# Autodesk Inventor assembly: 000-base_wheel-v3
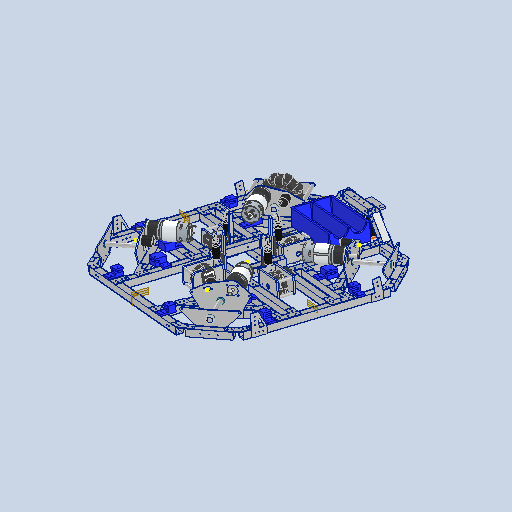
[picture p0: Inventor's stored thumbnail of the model, 512x512]
Saved by Autodesk Inventor 2025.2 (Build 292293000, 293)
## iProperties
Created: 2025-04-01
Part Number: 000-base_wheel-v3
Document SubType Name: Assembly
Designer: haruy
Author: haruy
## Documents named in this file (28)
- C:\Users\haruy\Documents\ロボコン\NHK2025\cad\nagahisa\base_weel\000-base_wheel-v3.iam
- C:\Users\haruy\Documents\ロボコン\NHK2025\cad\nagahisa\base_weel\base_weel-v3-ASP-Base.ipt
- C:\Users\haruy\Documents\ロボコン\NHK2025\cad\nagahisa\base_weel\base_weel-v3-Plate-1.ipt
- C:\Users\haruy\Documents\ロボコン\NHK2025\cad\nagahisa\base_weel\base_weel-v3-Plate-2.ipt
- C:\Users\haruy\Documents\ロボコン\NHK2025\cad\nagahisa\base_weel\takagi_weel\Workspaces\作業スペース\takagi\omuni_wheel_ver3.0\parts\frequently used parts\モーター\RS775\rs775_4.iam
- C:\Users\haruy\Documents\ロボコン\NHK2025\cad\000_parts\エンコーダー\encoder v2.ipt
- C:\Users\haruy\Documents\ロボコン\NHK2025\cad\nagahisa\odom\odom_v1_Plate_5.ipt
- C:\Users\haruy\Documents\ロボコン\NHK2025\cad\nagahisa\odom\000-odom-v1.iam
- C:\Users\haruy\Documents\ロボコン\NHK2025\cad\nagahisa\odom\odom_v1_Plate_6.ipt
- C:\Users\haruy\Documents\ロボコン\NHK2025\cad\nagahisa\base_weel\base_weel-v3-Plate-3.ipt
- C:\Users\haruy\Documents\ロボコン\NHK2025\cad\nagahisa\base_weel\base_weel-v3-Plate-4.ipt
- C:\Users\haruy\Documents\ロボコン\NHK2025\cad\nagahisa\base_weel\base_weel-v3-Plate-5.ipt
- C:\Users\haruy\Documents\ロボコン\NHK2025\cad\nagahisa\base_weel\base_weel-v3-Plate-6.ipt
- C:\Users\haruy\Documents\ロボコン\NHK2025\cad\nagahisa\dribl\R2-Rzvector\TH22_bearing_12_18_19.5_sn.ipt
- C:\Users\haruy\Documents\ロボコン\NHK2025\cad\nagahisa\base_weel\SCBRJ12-15.iam
- C:\Users\haruy\Documents\ロボコン\NHK2025\cad\nagahisa\base_weel\base_weel-v3-Shaft-1.ipt
- C:\Users\haruy\Documents\ロボコン\NHK2025\cad\nagahisa\base_weel\takagi_weel\Workspaces\作業スペース\takagi\omuni_wheel_ver3.0\parts\frequently used parts\タイヤ\omni wheel\100mm wheel\100mm omuniwheel_MIR1.iam
- C:\Users\haruy\Documents\ロボコン\NHK2025\cad\nagahisa\base_weel\base_weel-v3-Shaft-2.ipt
- C:\Users\haruy\Documents\ロボコン\NHK2025\cad\nagahisa\base_weel\base_weel-v3-Plate-7.ipt
- C:\Users\haruy\Documents\ロボコン\NHK2025\cad\nagahisa\base_weel\roja-v1-3DP-lipo-box.ipt
- C:\Users\haruy\Documents\ロボコン\NHK2025\cad\nagahisa\base_weel\base_weel-v3-3DP-1.ipt
- C:\Users\haruy\Documents\ロボコン\NHK2025\cad\nagahisa\base_weel\base_weel-v3-3DP-2.ipt
- C:\Users\haruy\Documents\ロボコン\NHK2025\cad\nagahisa\base_weel\base_weel-v3-Plate-8.ipt
- C:\Users\haruy\Documents\ロボコン\NHK2025\cad\000_parts\センサー\LiDAR_true.iam
- C:\Users\haruy\Documents\ロボコン\NHK2025\cad\nagahisa\base_weel\base_weel-v3-Plate-9.ipt
- C:\Users\haruy\Documents\ロボコン\NHK2025\cad\nagahisa\base_weel\base_weel-v3-Plate-10.ipt
- C:\Users\haruy\Documents\ロボコン\NHK2025\cad\nagahisa\dribl\dribl-v1-Plate-9.ipt
- C:\Users\haruy\Documents\ロボコン\NHK2025\cad\nagahisa\dribl\dribl-v3-Plate-5.ipt
## Components (93 placed, 27 different names)
1. base_weel-v3-ASP-Base:1 — 挿入:1, 挿入:2, 挿入:3, 挿入:4, 挿入:5, 挿入:6, 挿入:7, 挿入:8, 挿入:9, 挿入:10, 挿入:11, 挿入:12, 挿入:13, 挿入:14, 挿入:15, 挿入:16, 挿入:25, 挿入:26, 挿入:27, 挿入:28, 挿入:35, 挿入:36, 挿入:37, 挿入:38, 挿入:45, 挿入:46, 挿入:47, 挿入:48, 挿入:49, 挿入:50, 挿入:51, 挿入:52, 挿入:53, 挿入:54, 挿入:55, 挿入:56, 挿入:57, 挿入:58, 挿入:59, 挿入:60, 挿入:61, 挿入:62, 挿入:63, 挿入:64, 挿入:65, 挿入:66, 挿入:67, 挿入:68, 挿入:69, 挿入:70, 挿入:71, 挿入:72, 挿入:73, 挿入:74, 挿入:75, 挿入:76, 挿入:77, 挿入:78, 挿入:79, 挿入:80, 挿入:81, 挿入:82, 挿入:87, 挿入:88, 挿入:89, 挿入:90, 挿入:91, 挿入:92, 挿入:93, 挿入:94, 挿入:95, 挿入:96, 挿入:97, 挿入:98, 挿入:99, 挿入:100, 角度:1, 挿入:124, 挿入:125, 挿入:126, 挿入:127, 挿入:128, 挿入:129, 挿入:130, 挿入:131, 挿入:132, 挿入:133, 挿入:134, 挿入:135, 挿入:136, 挿入:137, 挿入:138, 挿入:139, 挿入:140, 挿入:141, 挿入:142, 挿入:143, 挿入:146, 挿入:147, 挿入:148, 挿入:149, 挿入:150, 挿入:151, 挿入:152, 挿入:153, 挿入:154, 挿入:155, 挿入:156, 挿入:157, 挿入:158, 挿入:159, 挿入:160, 挿入:161
2. base_weel-v3-Plate-1:1 — 挿入:1, 挿入:2, 挿入:108
3. base_weel-v3-Plate-1:2 — 挿入:3, 挿入:4, 挿入:105
4. base_weel-v3-Plate-1:3 — 挿入:7, 挿入:8, 挿入:101
5. base_weel-v3-Plate-1:4 — 挿入:5, 挿入:6, 挿入:103
6. base_weel-v3-Plate-2:1 — 挿入:9, 挿入:10, 挿入:17, 挿入:23, 挿入:104
7. base_weel-v3-Plate-2:2 — 挿入:11, 挿入:12, 挿入:20, 挿入:21, 挿入:107
8. base_weel-v3-Plate-2:3 — 挿入:13, 挿入:14, 挿入:18, 挿入:24, 挿入:102, 挿入:122, 挿入:123
9. base_weel-v3-Plate-2:4 — 挿入:15, 挿入:16, 挿入:19, 挿入:22, 挿入:106
10. rs775_4:1 [sub-assembly] — 挿入:17
11. rs775_4:2 [sub-assembly] — 挿入:18
12. rs775_4:3 [sub-assembly] — 挿入:19
13. rs775_4:4 [sub-assembly] — 挿入:20
14. encoder v2:1 — 挿入:21
15. encoder v2:2 — 挿入:22
16. encoder v2:3 — 挿入:23
17. encoder v2:4 — 挿入:24
18. odom_v1_Plate_5:1 — 挿入:26, 挿入:28, 挿入:29, 挿入:30, 挿入:31
19. odom_v1_Plate_5:2 — 挿入:25, 挿入:27, 挿入:32, 挿入:33, 挿入:34
20. 000-odom-v1:1 [sub-assembly] — 挿入:29, 挿入:30, 挿入:31
21. 000-odom-v1:2 [sub-assembly] — 挿入:32, 挿入:33, 挿入:34
22. odom_v1_Plate_6:1 — 挿入:35, 挿入:36, 挿入:39, 挿入:40, 挿入:41
23. odom_v1_Plate_6:2 — 挿入:37, 挿入:38, 挿入:42, 挿入:43, 挿入:44
24. 000-odom-v1:3 [sub-assembly] — 挿入:39, 挿入:40, 挿入:41
25. 000-odom-v1:4 [sub-assembly] — 挿入:42, 挿入:43, 挿入:44
26. base_weel-v3-Plate-3:1 — 挿入:45, 挿入:46
27. base_weel-v3-Plate-3:2 — 挿入:47, 挿入:48
28. base_weel-v3-Plate-3:3 — 挿入:49, 挿入:50
29. base_weel-v3-Plate-3:4 — 挿入:51, 挿入:52
30. base_weel-v3-Plate-3:5 — 挿入:53, 挿入:54
31. base_weel-v3-Plate-3:6 — 挿入:57, 挿入:58
32. base_weel-v3-Plate-3:7 — 挿入:59, 挿入:60
33. base_weel-v3-Plate-3:8 — 挿入:55, 挿入:56
34. base_weel-v3-Plate-4:1 — 挿入:61, 挿入:62
35. base_weel-v3-Plate-4:2 — 挿入:63, 挿入:64
36. base_weel-v3-Plate-4:3 — 挿入:67, 挿入:68
37. base_weel-v3-Plate-4:4 — 挿入:65, 挿入:66
38. base_weel-v3-Plate-4:5 — 挿入:71, 挿入:72
39. base_weel-v3-Plate-4:6 — 挿入:73, 挿入:74
40. base_weel-v3-Plate-4:7 — 挿入:69, 挿入:70
41. base_weel-v3-Plate-4:8 — 挿入:75, 挿入:76
42. base_weel-v3-Plate-5:1 — 挿入:77, 挿入:78
43. base_weel-v3-Plate-5:2 — 挿入:79, 挿入:80
44. base_weel-v3-Plate-5:3 — 挿入:81, 挿入:82
45. base_weel-v3-Plate-5:6 — 挿入:87, 挿入:88
46. base_weel-v3-Plate-5:7 — 挿入:89, 挿入:90
47. base_weel-v3-Plate-5:8 — 挿入:91, 挿入:92
48. base_weel-v3-Plate-6:1 — 挿入:93, 挿入:94
49. base_weel-v3-Plate-6:2 — 挿入:95, 挿入:96
50. base_weel-v3-Plate-6:3 — 挿入:97, 挿入:98
51. base_weel-v3-Plate-6:4 — 挿入:99, 挿入:100
52. TH22_bearing_12_18_19.5_sn:1 — 挿入:101, 挿入:113, 挿入:121
53. TH22_bearing_12_18_19.5_sn:2 — 挿入:102, 挿入:114
54. TH22_bearing_12_18_19.5_sn:3 — 挿入:104, 挿入:115
55. TH22_bearing_12_18_19.5_sn:4 — 挿入:103, 挿入:116
56. TH22_bearing_12_18_19.5_sn:5 — 挿入:105, 挿入:109
57. TH22_bearing_12_18_19.5_sn:6 — 挿入:107, 挿入:112
58. TH22_bearing_12_18_19.5_sn:7 — 挿入:106, 挿入:110
59. TH22_bearing_12_18_19.5_sn:8 — 挿入:108, 挿入:111
60. SCBRJ12-15:1 [sub-assembly] — 挿入:116, 挿入:120
61. SCBRJ12-15:2 [sub-assembly] — 挿入:112
62. SCBRJ12-15:3 [sub-assembly] — 挿入:115
63. SCBRJ12-15:4 [sub-assembly] — 挿入:109, 挿入:117
64. SCBRJ12-15:5 [sub-assembly] — 挿入:114
65. SCBRJ12-15:6 [sub-assembly] — 挿入:110
66. SCBRJ12-15:7 [sub-assembly] — 挿入:113, 挿入:119
67. SCBRJ12-15:8 [sub-assembly] — 挿入:111, 挿入:118
68. base_weel-v3-Shaft-1:1 — 挿入:117
69. base_weel-v3-Shaft-1:2 — 挿入:118
70. base_weel-v3-Shaft-1:3 — 挿入:119
71. base_weel-v3-Shaft-1:4 — 挿入:120
72. 100mm omuniwheel_MIR1:1 [sub-assembly] — 挿入:121, 角度:1
73. base_weel-v3-Shaft-2:1 — 挿入:122
74. base_weel-v3-Shaft-2:2 — 挿入:123
75. base_weel-v3-Plate-7:1 — 挿入:124, 挿入:125
76. base_weel-v3-Plate-7:2 — 挿入:126, 挿入:127
77. roja-v1-3DP-lipo-box:1 — 挿入:128, 挿入:129
78. base_weel-v3-3DP-1:2 — 挿入:130, 挿入:131
79. base_weel-v3-3DP-1:3 — 挿入:134, 挿入:135
80. base_weel-v3-3DP-1:6 — 挿入:132, 挿入:133
81. base_weel-v3-3DP-2:1 — 挿入:136, 挿入:137
82. base_weel-v3-3DP-2:2 — 挿入:138, 挿入:139
83. base_weel-v3-3DP-2:3 — 挿入:140, 挿入:141
84. base_weel-v3-Plate-8:1 — 挿入:142, 挿入:143, 挿入:144, 挿入:145
85. LiDAR_true:1 [sub-assembly] — 挿入:144, 挿入:145
86. base_weel-v3-Plate-9:1 — 挿入:146, 挿入:147
87. base_weel-v3-Plate-9:2 — 挿入:148, 挿入:149
88. base_weel-v3-Plate-10:1 — 挿入:150, 挿入:151
89. base_weel-v3-Plate-10:2 — 挿入:152, 挿入:153
90. dribl-v1-Plate-9:1 — 挿入:156, 挿入:157
91. dribl-v1-Plate-9:2 — 挿入:154, 挿入:155
92. dribl-v3-Plate-5:1 — 挿入:158, 挿入:159
93. dribl-v3-Plate-5:2 — 挿入:160, 挿入:161
## Relationships (158: Insert 157, Angle 1)
- 挿入:1 [Insert]: base_weel-v3-ASP-Base:1 ↔ base_weel-v3-Plate-1:1
- 挿入:2 [Insert]: base_weel-v3-ASP-Base:1 ↔ base_weel-v3-Plate-1:1
- 挿入:3 [Insert]: base_weel-v3-ASP-Base:1 ↔ base_weel-v3-Plate-1:2
- 挿入:4 [Insert]: base_weel-v3-ASP-Base:1 ↔ base_weel-v3-Plate-1:2
- 挿入:5 [Insert]: base_weel-v3-ASP-Base:1 ↔ base_weel-v3-Plate-1:4
- 挿入:6 [Insert]: base_weel-v3-ASP-Base:1 ↔ base_weel-v3-Plate-1:4
- 挿入:7 [Insert]: base_weel-v3-ASP-Base:1 ↔ base_weel-v3-Plate-1:3
- 挿入:8 [Insert]: base_weel-v3-ASP-Base:1 ↔ base_weel-v3-Plate-1:3
- 挿入:9 [Insert]: base_weel-v3-ASP-Base:1 ↔ base_weel-v3-Plate-2:1
- 挿入:10 [Insert]: base_weel-v3-ASP-Base:1 ↔ base_weel-v3-Plate-2:1
- 挿入:11 [Insert]: base_weel-v3-ASP-Base:1 ↔ base_weel-v3-Plate-2:2
- 挿入:12 [Insert]: base_weel-v3-ASP-Base:1 ↔ base_weel-v3-Plate-2:2
- 挿入:13 [Insert]: base_weel-v3-ASP-Base:1 ↔ base_weel-v3-Plate-2:3
- 挿入:14 [Insert]: base_weel-v3-ASP-Base:1 ↔ base_weel-v3-Plate-2:3
- 挿入:15 [Insert]: base_weel-v3-ASP-Base:1 ↔ base_weel-v3-Plate-2:4
- 挿入:16 [Insert]: base_weel-v3-ASP-Base:1 ↔ base_weel-v3-Plate-2:4
- 挿入:17 [Insert]: base_weel-v3-Plate-2:1 ↔ rs775_4:1
- 挿入:18 [Insert]: base_weel-v3-Plate-2:3 ↔ rs775_4:2
- 挿入:19 [Insert]: base_weel-v3-Plate-2:4 ↔ rs775_4:3
- 挿入:20 [Insert]: base_weel-v3-Plate-2:2 ↔ rs775_4:4
- 挿入:21 [Insert]: base_weel-v3-Plate-2:2 ↔ encoder v2:1
- 挿入:22 [Insert]: base_weel-v3-Plate-2:4 ↔ encoder v2:2
- 挿入:23 [Insert]: base_weel-v3-Plate-2:1 ↔ encoder v2:3
- 挿入:24 [Insert]: base_weel-v3-Plate-2:3 ↔ encoder v2:4
- 挿入:25 [Insert]: base_weel-v3-ASP-Base:1 ↔ odom_v1_Plate_5:2
- 挿入:26 [Insert]: base_weel-v3-ASP-Base:1 ↔ odom_v1_Plate_5:1
- 挿入:27 [Insert]: base_weel-v3-ASP-Base:1 ↔ odom_v1_Plate_5:2
- 挿入:28 [Insert]: base_weel-v3-ASP-Base:1 ↔ odom_v1_Plate_5:1
- 挿入:29 [Insert]: odom_v1_Plate_5:1 ↔ 000-odom-v1:1
- 挿入:30 [Insert]: odom_v1_Plate_5:1 ↔ 000-odom-v1:1
- 挿入:31 [Insert]: odom_v1_Plate_5:1 ↔ 000-odom-v1:1
- 挿入:32 [Insert]: odom_v1_Plate_5:2 ↔ 000-odom-v1:2
- 挿入:33 [Insert]: odom_v1_Plate_5:2 ↔ 000-odom-v1:2
- 挿入:34 [Insert]: odom_v1_Plate_5:2 ↔ 000-odom-v1:2
- 挿入:35 [Insert]: base_weel-v3-ASP-Base:1 ↔ odom_v1_Plate_6:1
- 挿入:36 [Insert]: base_weel-v3-ASP-Base:1 ↔ odom_v1_Plate_6:1
- 挿入:37 [Insert]: base_weel-v3-ASP-Base:1 ↔ odom_v1_Plate_6:2
- 挿入:38 [Insert]: base_weel-v3-ASP-Base:1 ↔ odom_v1_Plate_6:2
- 挿入:39 [Insert]: odom_v1_Plate_6:1 ↔ 000-odom-v1:3
- 挿入:40 [Insert]: odom_v1_Plate_6:1 ↔ 000-odom-v1:3
- 挿入:41 [Insert]: odom_v1_Plate_6:1 ↔ 000-odom-v1:3
- 挿入:42 [Insert]: odom_v1_Plate_6:2 ↔ 000-odom-v1:4
- 挿入:43 [Insert]: odom_v1_Plate_6:2 ↔ 000-odom-v1:4
- 挿入:44 [Insert]: odom_v1_Plate_6:2 ↔ 000-odom-v1:4
- 挿入:45 [Insert]: base_weel-v3-ASP-Base:1 ↔ base_weel-v3-Plate-3:1
- 挿入:46 [Insert]: base_weel-v3-ASP-Base:1 ↔ base_weel-v3-Plate-3:1
- 挿入:47 [Insert]: base_weel-v3-ASP-Base:1 ↔ base_weel-v3-Plate-3:2
- 挿入:48 [Insert]: base_weel-v3-ASP-Base:1 ↔ base_weel-v3-Plate-3:2
- 挿入:49 [Insert]: base_weel-v3-ASP-Base:1 ↔ base_weel-v3-Plate-3:3
- 挿入:50 [Insert]: base_weel-v3-ASP-Base:1 ↔ base_weel-v3-Plate-3:3
- 挿入:51 [Insert]: base_weel-v3-ASP-Base:1 ↔ base_weel-v3-Plate-3:4
- 挿入:52 [Insert]: base_weel-v3-ASP-Base:1 ↔ base_weel-v3-Plate-3:4
- 挿入:53 [Insert]: base_weel-v3-ASP-Base:1 ↔ base_weel-v3-Plate-3:5
- 挿入:54 [Insert]: base_weel-v3-ASP-Base:1 ↔ base_weel-v3-Plate-3:5
- 挿入:55 [Insert]: base_weel-v3-ASP-Base:1 ↔ base_weel-v3-Plate-3:8
- 挿入:56 [Insert]: base_weel-v3-ASP-Base:1 ↔ base_weel-v3-Plate-3:8
- 挿入:57 [Insert]: base_weel-v3-ASP-Base:1 ↔ base_weel-v3-Plate-3:6
- 挿入:58 [Insert]: base_weel-v3-ASP-Base:1 ↔ base_weel-v3-Plate-3:6
- 挿入:59 [Insert]: base_weel-v3-ASP-Base:1 ↔ base_weel-v3-Plate-3:7
- 挿入:60 [Insert]: base_weel-v3-ASP-Base:1 ↔ base_weel-v3-Plate-3:7
- 挿入:61 [Insert]: base_weel-v3-ASP-Base:1 ↔ base_weel-v3-Plate-4:1
- 挿入:62 [Insert]: base_weel-v3-ASP-Base:1 ↔ base_weel-v3-Plate-4:1
- 挿入:63 [Insert]: base_weel-v3-ASP-Base:1 ↔ base_weel-v3-Plate-4:2
- 挿入:64 [Insert]: base_weel-v3-ASP-Base:1 ↔ base_weel-v3-Plate-4:2
- 挿入:65 [Insert]: base_weel-v3-ASP-Base:1 ↔ base_weel-v3-Plate-4:4
- 挿入:66 [Insert]: base_weel-v3-ASP-Base:1 ↔ base_weel-v3-Plate-4:4
- 挿入:67 [Insert]: base_weel-v3-ASP-Base:1 ↔ base_weel-v3-Plate-4:3
- 挿入:68 [Insert]: base_weel-v3-ASP-Base:1 ↔ base_weel-v3-Plate-4:3
- 挿入:69 [Insert]: base_weel-v3-ASP-Base:1 ↔ base_weel-v3-Plate-4:7
- 挿入:70 [Insert]: base_weel-v3-ASP-Base:1 ↔ base_weel-v3-Plate-4:7
- 挿入:71 [Insert]: base_weel-v3-ASP-Base:1 ↔ base_weel-v3-Plate-4:5
- 挿入:72 [Insert]: base_weel-v3-ASP-Base:1 ↔ base_weel-v3-Plate-4:5
- 挿入:73 [Insert]: base_weel-v3-ASP-Base:1 ↔ base_weel-v3-Plate-4:6
- 挿入:74 [Insert]: base_weel-v3-ASP-Base:1 ↔ base_weel-v3-Plate-4:6
- 挿入:75 [Insert]: base_weel-v3-ASP-Base:1 ↔ base_weel-v3-Plate-4:8
- 挿入:76 [Insert]: base_weel-v3-ASP-Base:1 ↔ base_weel-v3-Plate-4:8
- 挿入:77 [Insert]: base_weel-v3-ASP-Base:1 ↔ base_weel-v3-Plate-5:1
- 挿入:78 [Insert]: base_weel-v3-ASP-Base:1 ↔ base_weel-v3-Plate-5:1
- 挿入:79 [Insert]: base_weel-v3-ASP-Base:1 ↔ base_weel-v3-Plate-5:2
- 挿入:80 [Insert]: base_weel-v3-ASP-Base:1 ↔ base_weel-v3-Plate-5:2
- 挿入:81 [Insert]: base_weel-v3-ASP-Base:1 ↔ base_weel-v3-Plate-5:3
- 挿入:82 [Insert]: base_weel-v3-ASP-Base:1 ↔ base_weel-v3-Plate-5:3
- 挿入:87 [Insert]: base_weel-v3-ASP-Base:1 ↔ base_weel-v3-Plate-5:6
- 挿入:88 [Insert]: base_weel-v3-ASP-Base:1 ↔ base_weel-v3-Plate-5:6
- 挿入:89 [Insert]: base_weel-v3-ASP-Base:1 ↔ base_weel-v3-Plate-5:7
- 挿入:90 [Insert]: base_weel-v3-ASP-Base:1 ↔ base_weel-v3-Plate-5:7
- 挿入:91 [Insert]: base_weel-v3-ASP-Base:1 ↔ base_weel-v3-Plate-5:8
- 挿入:92 [Insert]: base_weel-v3-ASP-Base:1 ↔ base_weel-v3-Plate-5:8
- 挿入:93 [Insert]: base_weel-v3-ASP-Base:1 ↔ base_weel-v3-Plate-6:1
- 挿入:94 [Insert]: base_weel-v3-ASP-Base:1 ↔ base_weel-v3-Plate-6:1
- 挿入:95 [Insert]: base_weel-v3-ASP-Base:1 ↔ base_weel-v3-Plate-6:2
- 挿入:96 [Insert]: base_weel-v3-ASP-Base:1 ↔ base_weel-v3-Plate-6:2
- 挿入:97 [Insert]: base_weel-v3-ASP-Base:1 ↔ base_weel-v3-Plate-6:3
- 挿入:98 [Insert]: base_weel-v3-ASP-Base:1 ↔ base_weel-v3-Plate-6:3
- 挿入:99 [Insert]: base_weel-v3-ASP-Base:1 ↔ base_weel-v3-Plate-6:4
- 挿入:100 [Insert]: base_weel-v3-ASP-Base:1 ↔ base_weel-v3-Plate-6:4
- 挿入:101 [Insert]: base_weel-v3-Plate-1:3 ↔ TH22_bearing_12_18_19.5_sn:1
- 挿入:102 [Insert]: base_weel-v3-Plate-2:3 ↔ TH22_bearing_12_18_19.5_sn:2
- 挿入:103 [Insert]: base_weel-v3-Plate-1:4 ↔ TH22_bearing_12_18_19.5_sn:4
- 挿入:104 [Insert]: base_weel-v3-Plate-2:1 ↔ TH22_bearing_12_18_19.5_sn:3
- 挿入:105 [Insert]: base_weel-v3-Plate-1:2 ↔ TH22_bearing_12_18_19.5_sn:5
- 挿入:106 [Insert]: base_weel-v3-Plate-2:4 ↔ TH22_bearing_12_18_19.5_sn:7
- 挿入:107 [Insert]: base_weel-v3-Plate-2:2 ↔ TH22_bearing_12_18_19.5_sn:6
- 挿入:108 [Insert]: base_weel-v3-Plate-1:1 ↔ TH22_bearing_12_18_19.5_sn:8
- 挿入:109 [Insert]: TH22_bearing_12_18_19.5_sn:5 ↔ SCBRJ12-15:4
- 挿入:110 [Insert]: TH22_bearing_12_18_19.5_sn:7 ↔ SCBRJ12-15:6
- 挿入:111 [Insert]: TH22_bearing_12_18_19.5_sn:8 ↔ SCBRJ12-15:8
- 挿入:112 [Insert]: TH22_bearing_12_18_19.5_sn:6 ↔ SCBRJ12-15:2
- 挿入:113 [Insert]: TH22_bearing_12_18_19.5_sn:1 ↔ SCBRJ12-15:7
- 挿入:114 [Insert]: TH22_bearing_12_18_19.5_sn:2 ↔ SCBRJ12-15:5
- 挿入:115 [Insert]: TH22_bearing_12_18_19.5_sn:3 ↔ SCBRJ12-15:3
- 挿入:116 [Insert]: TH22_bearing_12_18_19.5_sn:4 ↔ SCBRJ12-15:1
- 挿入:117 [Insert] (-0.5 mm): SCBRJ12-15:4 ↔ base_weel-v3-Shaft-1:1
- 挿入:118 [Insert] (-0.5 mm): SCBRJ12-15:8 ↔ base_weel-v3-Shaft-1:2
- 挿入:119 [Insert] (-0.5 mm): SCBRJ12-15:7 ↔ base_weel-v3-Shaft-1:3
- 挿入:120 [Insert] (-0.5 mm): SCBRJ12-15:1 ↔ base_weel-v3-Shaft-1:4
- 挿入:121 [Insert] (-21.5 mm): TH22_bearing_12_18_19.5_sn:1 ↔ 100mm omuniwheel_MIR1:1
- 角度:1 [Angle] (180 deg): base_weel-v3-ASP-Base:1 ↔ 100mm omuniwheel_MIR1:1
- 挿入:122 [Insert]: base_weel-v3-Plate-2:3 ↔ base_weel-v3-Shaft-2:1
- 挿入:123 [Insert]: base_weel-v3-Plate-2:3 ↔ base_weel-v3-Shaft-2:2
- 挿入:124 [Insert]: base_weel-v3-ASP-Base:1 ↔ base_weel-v3-Plate-7:1
- 挿入:125 [Insert]: base_weel-v3-ASP-Base:1 ↔ base_weel-v3-Plate-7:1
- 挿入:126 [Insert]: base_weel-v3-ASP-Base:1 ↔ base_weel-v3-Plate-7:2
- 挿入:127 [Insert]: base_weel-v3-ASP-Base:1 ↔ base_weel-v3-Plate-7:2
- 挿入:128 [Insert]: base_weel-v3-ASP-Base:1 ↔ roja-v1-3DP-lipo-box:1
- 挿入:129 [Insert]: base_weel-v3-ASP-Base:1 ↔ roja-v1-3DP-lipo-box:1
- 挿入:130 [Insert]: base_weel-v3-ASP-Base:1 ↔ base_weel-v3-3DP-1:2
- 挿入:131 [Insert]: base_weel-v3-ASP-Base:1 ↔ base_weel-v3-3DP-1:2
- 挿入:132 [Insert]: base_weel-v3-ASP-Base:1 ↔ base_weel-v3-3DP-1:6
- 挿入:133 [Insert]: base_weel-v3-ASP-Base:1 ↔ base_weel-v3-3DP-1:6
- 挿入:134 [Insert]: base_weel-v3-ASP-Base:1 ↔ base_weel-v3-3DP-1:3
- 挿入:135 [Insert]: base_weel-v3-ASP-Base:1 ↔ base_weel-v3-3DP-1:3
- 挿入:136 [Insert]: base_weel-v3-ASP-Base:1 ↔ base_weel-v3-3DP-2:1
- 挿入:137 [Insert]: base_weel-v3-ASP-Base:1 ↔ base_weel-v3-3DP-2:1
- 挿入:138 [Insert]: base_weel-v3-ASP-Base:1 ↔ base_weel-v3-3DP-2:2
- 挿入:139 [Insert]: base_weel-v3-ASP-Base:1 ↔ base_weel-v3-3DP-2:2
- 挿入:140 [Insert]: base_weel-v3-ASP-Base:1 ↔ base_weel-v3-3DP-2:3
- 挿入:141 [Insert]: base_weel-v3-ASP-Base:1 ↔ base_weel-v3-3DP-2:3
- 挿入:142 [Insert]: base_weel-v3-ASP-Base:1 ↔ base_weel-v3-Plate-8:1
- 挿入:143 [Insert]: base_weel-v3-ASP-Base:1 ↔ base_weel-v3-Plate-8:1
- 挿入:144 [Insert]: base_weel-v3-Plate-8:1 ↔ LiDAR_true:1
- 挿入:145 [Insert]: base_weel-v3-Plate-8:1 ↔ LiDAR_true:1
- 挿入:146 [Insert]: base_weel-v3-ASP-Base:1 ↔ base_weel-v3-Plate-9:1
- 挿入:147 [Insert]: base_weel-v3-ASP-Base:1 ↔ base_weel-v3-Plate-9:1
- 挿入:148 [Insert]: base_weel-v3-ASP-Base:1 ↔ base_weel-v3-Plate-9:2
- 挿入:149 [Insert]: base_weel-v3-ASP-Base:1 ↔ base_weel-v3-Plate-9:2
- 挿入:150 [Insert]: base_weel-v3-ASP-Base:1 ↔ base_weel-v3-Plate-10:1
- 挿入:151 [Insert]: base_weel-v3-ASP-Base:1 ↔ base_weel-v3-Plate-10:1
- 挿入:152 [Insert]: base_weel-v3-ASP-Base:1 ↔ base_weel-v3-Plate-10:2
- 挿入:153 [Insert]: base_weel-v3-ASP-Base:1 ↔ base_weel-v3-Plate-10:2
- 挿入:154 [Insert]: base_weel-v3-ASP-Base:1 ↔ dribl-v1-Plate-9:2
- 挿入:155 [Insert]: base_weel-v3-ASP-Base:1 ↔ dribl-v1-Plate-9:2
- 挿入:156 [Insert]: base_weel-v3-ASP-Base:1 ↔ dribl-v1-Plate-9:1
- 挿入:157 [Insert]: base_weel-v3-ASP-Base:1 ↔ dribl-v1-Plate-9:1
- 挿入:158 [Insert]: base_weel-v3-ASP-Base:1 ↔ dribl-v3-Plate-5:1
- 挿入:159 [Insert]: base_weel-v3-ASP-Base:1 ↔ dribl-v3-Plate-5:1
- 挿入:160 [Insert]: base_weel-v3-ASP-Base:1 ↔ dribl-v3-Plate-5:2
- 挿入:161 [Insert]: base_weel-v3-ASP-Base:1 ↔ dribl-v3-Plate-5:2
